# Autodesk Inventor assembly: lab view of cryostat
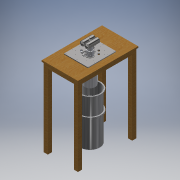
[picture p0: Inventor's stored thumbnail of the model, 180x180]
Saved by Autodesk Inventor 2018 (Build 220112000, 112)
## iProperties
Created: 2018-10-18
Part Number: lab view of cryostat
Document SubType Name: Assembly
Designer: freyja
Author: freyja
## Documents named in this file (3)
- C:\Users\freyja\Documents\Cryorefrigerator\CAD\lab view of cryostat.iam
- C:\Users\freyja\Documents\Cryorefrigerator\CAD\table.ipt
- C:\Users\freyja\Documents\Cryorefrigerator\CAD\mini Cryostat FOOT3.iam
## Components (2 placed, 2 different names)
1. table:1 — Mate:1, Angle:1, Mate:2
2. mini Cryostat FOOT3:1 [sub-assembly] — Mate:1, Angle:1, Mate:2
## Relationships (3: Mate 2, Angle 1)
- Mate:1: table:1 ↔ mini Cryostat FOOT3:1
- Angle:1 (0 deg): table:1 ↔ mini Cryostat FOOT3:1
- Mate:2: table:1 ↔ mini Cryostat FOOT3:1
